# Autodesk Inventor assembly: drive_shaft
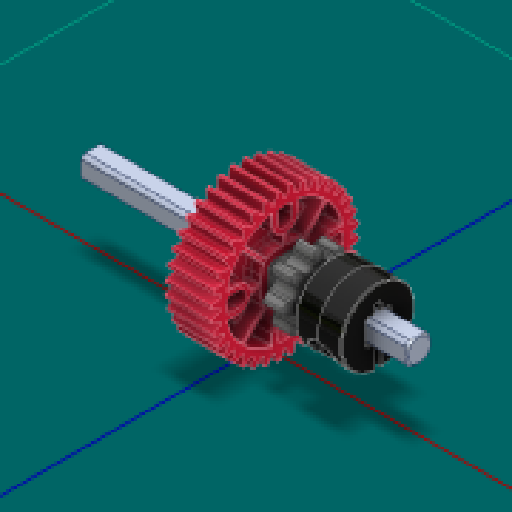
[picture p0: Inventor's stored thumbnail of the model, 512x512]
Saved by Autodesk Inventor 2025 (Build 290162000, 162)
## iProperties
Created: 2024-08-19
Part Number: drive_shaft
Document SubType Name: Assembly
Designer: averey
Author: averey
## Documents named in this file (10)
- C:\Users\avere\vex_robotics_high_stakes\hardware\cad\ATLAS\tower\intake_gearbox\drive_shaft_bottom.iam
- C:\Users\avere\vex_robotics_high_stakes\hardware\cad\VEX-CAD-Inventor\Motion\Gears\HS Gear\HS 36T Gear, No Insert.iam
- C:\Users\avere\vex_robotics_high_stakes\hardware\cad\VEX-CAD-Inventor\Motion\Gears\HS Gear.iam
- C:\Users\avere\vex_robotics_high_stakes\hardware\cad\VEX-CAD-Inventor\Motion\Shaft HS\HS Spacer\HSpacer .0625.ipt
- C:\Users\avere\vex_robotics_high_stakes\hardware\cad\VEX-CAD-Inventor\Motion\Shaft HS\HS Spacer.ipt
- C:\Users\avere\vex_robotics_high_stakes\hardware\cad\VEX-CAD-Inventor\Motion\Shaft HS\Shaft HS\Shaft HS 3.5 in.ipt
- C:\Users\avere\vex_robotics_high_stakes\hardware\cad\VEX-CAD-Inventor\Motion\Shaft HS\Shaft HS.ipt
- C:\Users\avere\vex_robotics_high_stakes\hardware\cad\VEX-CAD-Inventor\Motion\Sprockets\6P Sprocket\6P 8T Sprocket, No Insert.iam
- C:\Users\avere\vex_robotics_high_stakes\hardware\cad\VEX-CAD-Inventor\Motion\Sprockets\6P Sprocket.iam
- C:\Users\avere\vex_robotics_high_stakes\hardware\cad\VEX-CAD-Inventor\Motion\Shaft HS\HS Shaft Collar.ipt
## Components (5 placed, 5 different names)
1. HS 36T Gear, No Insert:1 [sub-assembly] — Insert:1, Insert:2, Insert:3
2. HSpacer .0625:1 — Insert:1
3. Shaft HS 3.5 in:1 — Insert:2
4. 6P 8T Sprocket, No Insert:1 [sub-assembly] — Insert:3, Insert:4
5. HS Shaft Collar:1 — Insert:4
## Relationships (4: Insert 4)
- Insert:1: HS 36T Gear, No Insert:1 ↔ HSpacer .0625:1
- Insert:2 (-36.5125 mm): HS 36T Gear, No Insert:1 ↔ Shaft HS 3.5 in:1
- Insert:3: HS 36T Gear, No Insert:1 ↔ 6P 8T Sprocket, No Insert:1
- Insert:4: 6P 8T Sprocket, No Insert:1 ↔ HS Shaft Collar:1
